# Autodesk Inventor assembly: ConPlanos
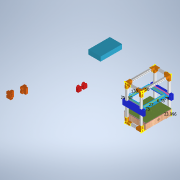
[picture p0: Inventor's stored thumbnail of the model, 180x180]
Saved by Autodesk Inventor 2022.6 (Build 266554000, 554)
## iProperties
Created: 2025-02-25
Part Number: ConPlanos
Document SubType Name: Assembly
Designer: Johan Gutiérrez
Author: Johan Gutiérrez
## Documents named in this file (15)
- D:\RutasNew\Desktop\Termoformadora\ConPlanos.iam
- D:\RutasNew\Desktop\Termoformadora\MADERA.ipt
- D:\RutasNew\Desktop\Termoformadora\Fomi.ipt
- D:\RutasNew\Desktop\Termoformadora\rejilla.ipt
- D:\RutasNew\Desktop\Termoformadora\esquina20mm.ipt
- D:\RutasNew\Desktop\Termoformadora\Perfil400mm.ipt
- D:\RutasNew\Desktop\Termoformadora\Travesaño.ipt
- D:\RutasNew\Desktop\Termoformadora\Tapa Inferior.ipt
- D:\RutasNew\Desktop\Termoformadora\Tapa Superior.ipt
- D:\RutasNew\Desktop\Termoformadora\REDONDA.ipt
- D:\RutasNew\Desktop\Termoformadora\Pestaña.ipt
- D:\RutasNew\Desktop\Termoformadora\Lamina Superior.ipt
- D:\RutasNew\Desktop\Termoformadora\Codo.ipt
- D:\RutasNew\Desktop\Termoformadora\Perfil146mm.ipt
- D:\RutasNew\Desktop\Termoformadora\Perfil300mm.ipt
## Components (34 placed, 14 different names)
1. MADERA:2 — Coincidencia:1, Nivelación:1, Nivelación:2, Nivelación:3, Nivelación:4, Coincidencia:3, Coincidencia:4, Coincidencia:9, Coincidencia:10, Coincidencia:11, Coincidencia:12, Coincidencia:13, Coincidencia:14
2. Fomi:1 — Coincidencia:1, Nivelación:1, Nivelación:2, Coincidencia:2
3. rejilla:1 — Coincidencia:2, Nivelación:3, Nivelación:4
4. Perfil400mm:1 — Coincidencia:5, Coincidencia:6, Coincidencia:19, Coincidencia:21, Coincidencia:24, Coincidencia:25
5. Travesaño:1 — Coincidencia:5, Coincidencia:6, Coincidencia:7, Coincidencia:8, Nivelación:5, Coincidencia:29, Nivelación:11
6. esquina20mm:1 — Coincidencia:3, Coincidencia:4
7. Perfil400mm:2 — Coincidencia:7, Coincidencia:8, Coincidencia:20, Coincidencia:26, Nivelación:10
8. esquina20mm:4 — Coincidencia:9, Coincidencia:10
9. esquina20mm:5 — Coincidencia:11, Coincidencia:12
10. esquina20mm:6 — Coincidencia:13, Coincidencia:14
11. Travesaño:2 — Coincidencia:15, Coincidencia:16, Coincidencia:17, Coincidencia:18, Nivelación:5, Coincidencia:30, Nivelación:12
12. Perfil400mm:3 — Coincidencia:15, Coincidencia:16, Coincidencia:27, Coincidencia:28
13. Perfil400mm:4 — Coincidencia:17, Coincidencia:18, Coincidencia:22, Coincidencia:23, Nivelación:13
14. esquina20mm:7 — Coincidencia:19, Nivelación:6, Nivelación:7
15. esquina20mm:8 — Nivelación:6, Nivelación:7, Nivelación:8, Nivelación:9
16. esquina20mm:10 — Coincidencia:20
17. Tapa Superior:1 — Coincidencia:33, Nivelación:15, Coincidencia:34
18. REDONDA:1
19. REDONDA:2
20. Pestaña:1 — Coincidencia:30, Nivelación:12, Nivelación:13, Coincidencia:31, Nivelación:14, Coincidencia:32
21. Pestaña:2 — Coincidencia:29, Nivelación:10, Nivelación:11
22. Lamina Superior:1
23. Codo:1
24. Codo:2
25. esquina20mm:11 — Nivelación:8, Nivelación:9
26. Perfil146mm:1 — Coincidencia:21
27. Perfil146mm:2 — Coincidencia:23
28. Perfil300mm:1 — Coincidencia:24
29. Perfil300mm:2 — Coincidencia:22
30. Perfil146mm:3 — Coincidencia:25
31. Perfil146mm:4 — Coincidencia:27
32. Perfil300mm:3 — Coincidencia:26
33. Perfil300mm:4 — Coincidencia:28
34. Tapa Inferior:1 — Coincidencia:31, Nivelación:14, Coincidencia:32, Coincidencia:33, Nivelación:15, Coincidencia:34
## Relationships (49: Mate 34, Flush 15)
- Coincidencia:1 [Mate]: MADERA:2 ↔ Fomi:1
- Nivelación:1 [Flush]: MADERA:2 ↔ Fomi:1
- Nivelación:2 [Flush]: MADERA:2 ↔ Fomi:1
- Coincidencia:2 [Mate]: Fomi:1 ↔ rejilla:1
- Nivelación:3 [Flush]: MADERA:2 ↔ rejilla:1
- Nivelación:4 [Flush]: MADERA:2 ↔ rejilla:1
- Coincidencia:3 [Mate]: MADERA:2 ↔ esquina20mm:1
- Coincidencia:4 [Mate]: MADERA:2 ↔ esquina20mm:1
- Coincidencia:5 [Mate]: Perfil400mm:1 ↔ Travesaño:1
- Coincidencia:6 [Mate]: Perfil400mm:1 ↔ Travesaño:1
- Coincidencia:7 [Mate]: Travesaño:1 ↔ Perfil400mm:2
- Coincidencia:8 [Mate]: Travesaño:1 ↔ Perfil400mm:2
- Coincidencia:9 [Mate]: MADERA:2 ↔ esquina20mm:4
- Coincidencia:10 [Mate]: MADERA:2 ↔ esquina20mm:4
- Coincidencia:11 [Mate]: MADERA:2 ↔ esquina20mm:5
- Coincidencia:12 [Mate]: MADERA:2 ↔ esquina20mm:5
- Coincidencia:13 [Mate]: MADERA:2 ↔ esquina20mm:6
- Coincidencia:14 [Mate]: MADERA:2 ↔ esquina20mm:6
- Coincidencia:15 [Mate]: Travesaño:2 ↔ Perfil400mm:3
- Coincidencia:16 [Mate]: Travesaño:2 ↔ Perfil400mm:3
- Coincidencia:17 [Mate]: Travesaño:2 ↔ Perfil400mm:4
- Coincidencia:18 [Mate]: Travesaño:2 ↔ Perfil400mm:4
- Nivelación:5 [Flush]: Travesaño:1 ↔ Travesaño:2
- Coincidencia:19 [Mate]: Perfil400mm:1 ↔ esquina20mm:7
- Coincidencia:20 [Mate]: Perfil400mm:2 ↔ esquina20mm:10
- Nivelación:6 [Flush]: esquina20mm:7 ↔ esquina20mm:8
- Nivelación:7 [Flush]: esquina20mm:7 ↔ esquina20mm:8
- Nivelación:8 [Flush]: esquina20mm:8 ↔ esquina20mm:11
- Nivelación:9 [Flush]: esquina20mm:8 ↔ esquina20mm:11
- Coincidencia:21 [Mate]: Perfil400mm:1 ↔ Perfil146mm:1
- Coincidencia:22 [Mate]: Perfil400mm:4 ↔ Perfil300mm:2
- Coincidencia:23 [Mate]: Perfil400mm:4 ↔ Perfil146mm:2
- Coincidencia:24 [Mate]: Perfil400mm:1 ↔ Perfil300mm:1
- Coincidencia:25 [Mate]: Perfil400mm:1 ↔ Perfil146mm:3
- Coincidencia:26 [Mate]: Perfil400mm:2 ↔ Perfil300mm:3
- Coincidencia:27 [Mate]: Perfil400mm:3 ↔ Perfil146mm:4
- Coincidencia:28 [Mate]: Perfil400mm:3 ↔ Perfil300mm:4
- Coincidencia:29 [Mate]: Travesaño:1 ↔ Pestaña:2
- Nivelación:10 [Flush]: Perfil400mm:2 ↔ Pestaña:2
- Nivelación:11 [Flush]: Travesaño:1 ↔ Pestaña:2
- Coincidencia:30 [Mate]: Travesaño:2 ↔ Pestaña:1
- Nivelación:12 [Flush]: Travesaño:2 ↔ Pestaña:1
- Nivelación:13 [Flush]: Perfil400mm:4 ↔ Pestaña:1
- Coincidencia:31 [Mate]: Pestaña:1 ↔ Tapa Inferior:1
- Nivelación:14 [Flush]: Pestaña:1 ↔ Tapa Inferior:1
- Coincidencia:32 [Mate]: Pestaña:1 ↔ Tapa Inferior:1
- Coincidencia:33 [Mate]: Tapa Superior:1 ↔ Tapa Inferior:1
- Nivelación:15 [Flush]: Tapa Superior:1 ↔ Tapa Inferior:1
- Coincidencia:34 [Mate]: Tapa Superior:1 ↔ Tapa Inferior:1
